# Autodesk Inventor assembly: 01-02 Servo_Gripper
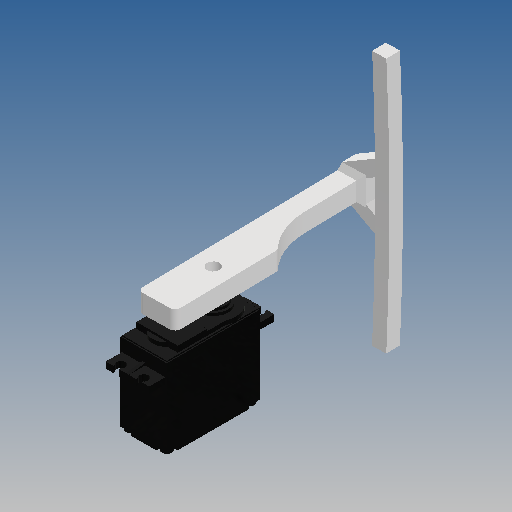
[picture p0: Inventor's stored thumbnail of the model, 512x512]
Saved by Autodesk Inventor 2026.2 (Build 302298000, 298)
## iProperties
Created: 2025-12-10
Part Number: 01-02 Servo_Gripper
Document SubType Name: Assembly
Designer: Schally
Author: Schally
## Documents named in this file (3)
- E:\06 Carologistics\02 Zeichnungen Greifer System\Gripper alt\01-02 Servo_Gripper.iam
- E:\06 Carologistics\02 Zeichnungen Greifer System\Gripper alt\01-02-01 Sandard-Servo.ipt
- E:\06 Carologistics\02 Zeichnungen Greifer System\Gripper alt\01-02-02 Gripper neu.ipt
## Components (2 placed, 2 different names)
1. 01-02-01 Sandard-Servo:1 — Passend:1
2. 01-02-02 Gripper neu:1 — Passend:1
## Relationships (1: Mate 1)
- Passend:1 [Mate]: 01-02-01 Sandard-Servo:1 ↔ 01-02-02 Gripper neu:1
